# Autodesk Inventor assembly: Big Shaft Motor Assembly
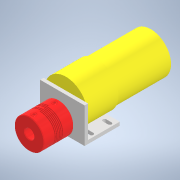
[picture p0: Inventor's stored thumbnail of the model, 180x180]
Saved by Autodesk Inventor 2022 (Build 260153000, 153)
## iProperties
Created: 2021-06-03
Part Number: Big Shaft Motor Assembly
Document SubType Name: Assembly
Designer: jrcol
Author: jrcol
## Documents named in this file (4)
- C:\Users\jrcol\Desktop\Solar-Lab-Files\Smart Drill\Big Shaft Motor Assembly.iam
- C:\Users\jrcol\Desktop\Solar-Lab-Files\Smart Drill\Big Motor.ipt
- C:\Users\jrcol\Desktop\Solar-Lab-Files\Smart Drill\Big shaft coupling.ipt
- C:\Users\jrcol\Desktop\Solar-Lab-Files\Smart Drill\Big Motor Bracket.ipt
## Components (3 placed, 3 different names)
1. Big Motor:1 — Mate:1, Mate:2, Mate:3, Mate:4, Mate:5
2. Big shaft coupling:1 — Mate:2, Mate:3, Mate:5
3. Big Motor Bracket:1 — Mate:1, Mate:4
## Relationships (5: Mate 5)
- Mate:1: Big Motor:1 ↔ Big Motor Bracket:1
- Mate:2: Big Motor:1 ↔ Big shaft coupling:1
- Mate:3: Big Motor:1 ↔ Big shaft coupling:1
- Mate:4: Big Motor:1 ↔ Big Motor Bracket:1
- Mate:5: Big Motor:1 ↔ Big shaft coupling:1
